# Autodesk Inventor assembly: Master
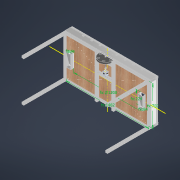
[picture p0: Inventor's stored thumbnail of the model, 180x180]
Saved by Autodesk Inventor 2021.4 (Build 254397000, 397)
## iProperties
Created: 2021-11-23
Part Number: Master
Document SubType Name: Assembly
Designer: jo_ki
Author: jo_ki
## Documents named in this file (35)
- D:\Repos\SmartSoccerTableCAD\Assemblies\Master.iam
- D:\Repos\SmartSoccerTableCAD\Parts\Beams\leg.ipt
- D:\Repos\SmartSoccerTableCAD\Parts\Beams\tallBeamLong.ipt
- D:\Repos\SmartSoccerTableCAD\Parts\Beams\tallBeamShort.ipt
- D:\Repos\SmartSoccerTableCAD\Parts\Beams\tallBeamLongInlet.ipt
- D:\Repos\SmartSoccerTableCAD\Parts\ballInlet\ballInletWheel.ipt
- D:\Repos\SmartSoccerTableCAD\Parts\Dimensions\Mastersketch.ipt
- D:\Repos\SmartSoccerTableCAD\Parts\Floors\GroundPlate.ipt
- D:\Repos\SmartSoccerTableCAD\Parts\Floors\glassPlate.ipt
- D:\Repos\SmartSoccerTableCAD\Parts\goalStructure\goalPanelFront.ipt
- D:\Repos\SmartSoccerTableCAD\Parts\goalStructure\goalPanelTop.ipt
- D:\Repos\SmartSoccerTableCAD\Parts\Beams\centerSupportBeam.ipt
- D:\Repos\SmartSoccerTableCAD\Import\stepper_am23hs0420-01\stepper_am23hs0420-01.iam
- D:\Repos\SmartSoccerTableCAD\Parts\Beams\centerAxleSupportBeam.ipt
- D:\Repos\SmartSoccerTableCAD\Parts\ballInlet\stepperMotorMount.ipt
- D:\Repos\SmartSoccerTableCAD\Parts\Beams\centerAxleSupportBeamHole.ipt
- D:\Repos\SmartSoccerTableCAD\Parts\ballInlet\axleMount\bearingShellInner.ipt
- D:\Repos\SmartSoccerTableCAD\Parts\ballInlet\axleMount\bearingShellOuter.ipt
- D:\Repos\SmartSoccerTableCAD\Parts\ballInlet\axleMount\centerAxleBearingSpacer.ipt
- C:\Users\jo_ki\OneDrive\Dokumente\Inventor\Content Center Files\R2021\en-US\DIN 625 SKF(4)\DIN 625 SKF - SKF 61800-2Z.ipt
- D:\Repos\SmartSoccerTableCAD\Parts\ballInlet\ballInletWheelAxle.ipt
- D:\Repos\SmartSoccerTableCAD\Parts\ballInlet\stepperToAxleConnector_1.ipt
- D:\Repos\SmartSoccerTableCAD\Parts\ballInlet\stepperToAxleConnector_2.ipt
- C:\Users\jo_ki\OneDrive\Dokumente\Inventor\Content Center Files\R2021\en-US\ISO 4762(2)\ISO 4762 - M3 x 6ISO.ipt
- C:\Users\jo_ki\OneDrive\Dokumente\Inventor\Content Center Files\R2021\en-US\ISO 4762(2)\ISO 4762 - M5 x 16ISO.ipt
- C:\Users\jo_ki\OneDrive\Dokumente\Inventor\Content Center Files\R2021\en-US\ISO 4035(2)\ISO 4035 - M10 - ISO.ipt
- C:\Users\jo_ki\OneDrive\Dokumente\Inventor\Content Center Files\R2021\en-US\ISO 7089\ISO 7089 - 10 - 140 HV(1).ipt
- D:\Repos\SmartSoccerTableCAD\Import\Nutenstein_8_St_M6\Nutenstein_8_St_M6.ipt
- C:\Users\jo_ki\OneDrive\Dokumente\Inventor\Content Center Files\R2021\en-US\ISO 4762(2)\ISO 4762 - M6 x 16ISO.ipt
- D:\Repos\SmartSoccerTableCAD\Parts\goalStructure\TorraumSeitenplatte.ipt
- D:\Repos\SmartSoccerTableCAD\Parts\goalStructure\TorraumSchrägeObenNEU.ipt
- D:\Repos\SmartSoccerTableCAD\Parts\goalStructure\TorraumHinten.ipt
- D:\Repos\SmartSoccerTableCAD\Parts\goalStructure\TorraumSchrägeUntenNEU.ipt
- D:\Repos\SmartSoccerTableCAD\Parts\goalStructure\TorraumSeiteBalleinwurf.ipt
- D:\Repos\SmartSoccerTableCAD\Parts\goalStructure\TorraumFrontKlein.ipt
## Components (53 placed, 33 different names)
1. glassPlate:1 — Mate:15, Mate:16, Flush:29, Mate:19, Mate:21
2. GroundPlate:1 — Mate:10, Mate:11, Mate:12, Mate:15, Flush:29, Mate:18, Mate:22, Mate:26, Mate:85
3. Nutenstein_8_St_M6:1 — Mate:80, Mate:81, Mate:82, Mate:83
4. ISO 4762 M6 x 16:1 — Mate:83, Mate:84
5. ISO 4762 M3 x 6:2 — Mate:62, Mate:63
6. ISO 4762 M3 x 6:3 — Mate:64, Mate:65
7. ISO 4762 M3 x 6:4 — Mate:66, Mate:67
8. ISO 4762 M5 x 16:1 — Mate:68, Mate:69
9. ISO 4762 M5 x 16:2 — Mate:70, Mate:71
10. ISO 4762 M5 x 16:3 — Mate:72, Mate:73
11. ISO 4762 M5 x 16:4 — Mate:74, Mate:75
12. ISO 7089 10:1 — Mate:76, Mate:77, Mate:79
13. ISO 4035 M10:1 — Mate:78, Mate:79, Angle:1
14. stepper_am23hs0420-01:1 [sub-assembly] — Flush:36, Flush:37, Mate:36, Mate:37, Mate:69, Mate:71, Mate:73, Mate:75
15. stepperMotorMount:1 — Mate:34, Mate:35, Flush:36, Flush:37, Mate:37, Mate:68, Mate:70, Mate:72, Mate:74, Mate:81, Mate:82, Mate:84
16. centerAxleSupportBeamHole:1 — Mate:38, Mate:39, Mate:40, Mate:41, Mate:50, Mate:51
17. bearingShellInner:1 — Mate:42, Mate:43, Mate:44, Mate:45, Mate:47
18. bearingShellOuter:1 — Mate:42, Mate:46, Mate:50, Mate:51
19. centerAxleBearingSpacer:1 — Mate:47, Mate:48, Mate:49
20. DIN 625 SKF- with two Z shields SKF 61800-2Z:1 — Mate:43, Mate:44, Mate:49
21. DIN 625 SKF- with two Z shields SKF 61800-2Z:2 — Mate:45, Mate:46, Mate:48
22. ballInletWheelAxle:1 — Mate:52, Mate:53, Mate:54, Mate:55, Mate:56, Mate:57, Mate:59, Mate:76, Mate:78, Angle:1
23. stepperToAxleConnector_1:1 — Flush:38, Mate:58, Mate:59, Mate:61, Mate:63, Mate:65, Mate:67
24. stepperToAxleConnector_2:1 — Mate:55, Mate:56, Mate:57, Flush:38, Mate:58, Mate:60, Mate:62, Mate:64, Mate:66
25. ISO 4762 M3 x 6:1 — Mate:60, Mate:61
26. centerSupportBeam:1 — Mate:29, Flush:32, Tangent:2, Mate:32, Flush:35, Mate:38
27. centerSupportBeam:2 — Mate:30, Flush:33, Tangent:1
28. centerAxleSupportBeam:1 — Mate:32, Flush:35, Mate:34, Mate:35, Mate:41, Mate:80
29. ballInletWheel:1 — Mate:9, Flush:17, Tangent:1, Tangent:2, Mate:36, Mate:39, Mate:40, Mate:52, Mate:53, Mate:54, Mate:77
30. leg:1 — Flush:1, Flush:23, Mate:14
31. leg:2 — Flush:14, Flush:15, Mate:8
32. leg:3 — Flush:3, Mate:13, Flush:21, Flush:22
33. leg:4 — Mate:6, Flush:12, Flush:13
34. tallBeamLong:1 — Flush:1, Flush:3, Mate:3, Mate:5, Mate:11, Flush:18, Flush:19, Flush:20, Mate:13, Flush:21, Mate:14, Mate:17, Mate:20, Mate:23, Mate:25
35. tallBeamShort:1 — Mate:5, Flush:15, Flush:16, Flush:20, Flush:22
36. tallBeamShort:2 — Mate:3, Flush:10, Mate:7, Flush:11, Flush:12, Mate:12, Flush:18, Flush:19, Flush:23
37. tallBeamLongInlet:1 — Mate:6, Flush:10, Mate:7, Flush:11, Flush:13, Flush:14, Flush:16, Mate:8, Mate:9, Flush:17, Mate:10, Mate:16, Mate:27, Mate:29, Flush:32, Mate:30, Flush:33
38. goalPanelFront:1 — Mate:17, Mate:18, Mate:19, Mate:26, Flush:31, Mate:28, Mate:86, Mate:88, Mate:90, Mate:99
39. TorraumSeitenplatte:1 — Mate:85, Mate:86, Mate:87, Mate:89, Flush:39, Flush:41
40. TorraumSchrägeObenNEU:1 — Mate:88, Mate:89, Mate:90, Mate:92
41. TorraumHinten:1 — Mate:91, Mate:92, Flush:39, Flush:40, Mate:93, Mate:94, Mate:95, Flush:42
42. TorraumSchrägeUntenNEU:1 — Flush:40, Mate:93, Mate:94, Mate:98
43. TorraumSeiteBalleinwurf:1 — Mate:95, Mate:97, Flush:42
44. TorraumFrontKlein:1 — Mate:98, Flush:41, Mate:99
45. goalPanelTop:1 — Mate:25, Mate:27, Flush:31, Mate:28, Mate:87, Mate:91, Mate:97
46. TorraumSeitenplatte:2 — Mate:110, Flush:45, Mate:111
47. TorraumFrontKlein:2 — Flush:43, Mate:106, Mate:107
48. TorraumHinten:2 — Mate:103, Mate:104, Mate:105, Mate:108, Flush:44, Mate:109, Mate:110, Flush:45, Mate:112
49. TorraumSchrägeObenNEU:2 — Mate:112, Mate:113, Mate:114
50. TorraumSchrägeUntenNEU:2 — Mate:108, Flush:44, Mate:109
51. TorraumSeiteBalleinwurf:2 — Mate:100, Mate:101, Mate:102, Mate:103, Mate:104, Mate:107, Mate:114
52. goalPanelTop:2 — Mate:23, Mate:24, Flush:30, Mate:101, Mate:105, Mate:111
53. goalPanelFront:2 — Mate:20, Mate:21, Mate:22, Mate:24, Flush:30, Mate:100, Mate:102, Flush:43, Mate:106, Mate:113
## Relationships (143: Mate 108, Flush 32, Tangent 2, Angle 1)
- Flush:1: leg:1 ↔ tallBeamLong:1
- Flush:3: leg:3 ↔ tallBeamLong:1
- Mate:3: tallBeamLong:1 ↔ tallBeamShort:2
- Mate:5: tallBeamLong:1 ↔ tallBeamShort:1
- Mate:6: leg:4 ↔ tallBeamLongInlet:1
- Flush:10: tallBeamShort:2 ↔ tallBeamLongInlet:1
- Mate:7: tallBeamShort:2 ↔ tallBeamLongInlet:1
- Flush:11: tallBeamShort:2 ↔ tallBeamLongInlet:1
- Flush:12: leg:4 ↔ tallBeamShort:2
- Flush:13: leg:4 ↔ tallBeamLongInlet:1
- Flush:14: leg:2 ↔ tallBeamLongInlet:1
- Flush:15: leg:2 ↔ tallBeamShort:1
- Flush:16: tallBeamShort:1 ↔ tallBeamLongInlet:1
- Mate:8: leg:2 ↔ tallBeamLongInlet:1
- Mate:9: ballInletWheel:1 ↔ tallBeamLongInlet:1
- Flush:17 (4.5 mm): ballInletWheel:1 ↔ tallBeamLongInlet:1
- Mate:10: GroundPlate:1 ↔ tallBeamLongInlet:1
- Mate:11 (-11 mm): GroundPlate:1 ↔ tallBeamLong:1
- Mate:12 (-11 mm): GroundPlate:1 ↔ tallBeamShort:2
- Flush:18: tallBeamLong:1 ↔ tallBeamShort:2
- Flush:19: tallBeamLong:1 ↔ tallBeamShort:2
- Flush:20: tallBeamLong:1 ↔ tallBeamShort:1
- Mate:13: leg:3 ↔ tallBeamLong:1
- Flush:21: leg:3 ↔ tallBeamLong:1
- Flush:22: leg:3 ↔ tallBeamShort:1
- Flush:23: leg:1 ↔ tallBeamShort:2
- Mate:14: leg:1 ↔ tallBeamLong:1
- Mate:15: glassPlate:1 ↔ GroundPlate:1
- Mate:16: glassPlate:1 ↔ tallBeamLongInlet:1
- Flush:29: glassPlate:1 ↔ GroundPlate:1
- Mate:17: tallBeamLong:1 ↔ goalPanelFront:1
- Mate:18: GroundPlate:1 ↔ goalPanelFront:1
- Mate:19: glassPlate:1 ↔ goalPanelFront:1
- Mate:20: tallBeamLong:1 ↔ goalPanelFront:2
- Mate:21: glassPlate:1 ↔ goalPanelFront:2
- Mate:22: GroundPlate:1 ↔ goalPanelFront:2
- Mate:23: tallBeamLong:1 ↔ goalPanelTop:2
- Mate:24: goalPanelTop:2 ↔ goalPanelFront:2
- Flush:30: goalPanelTop:2 ↔ goalPanelFront:2
- Mate:25: tallBeamLong:1 ↔ goalPanelTop:1
- Mate:26: GroundPlate:1 ↔ goalPanelFront:1
- Mate:27: tallBeamLongInlet:1 ↔ goalPanelTop:1
- Flush:31: goalPanelFront:1 ↔ goalPanelTop:1
- Mate:28: goalPanelFront:1 ↔ goalPanelTop:1
- Mate:29: centerSupportBeam:1 ↔ tallBeamLongInlet:1
- Flush:32: centerSupportBeam:1 ↔ tallBeamLongInlet:1
- Mate:30: centerSupportBeam:2 ↔ tallBeamLongInlet:1
- Flush:33: centerSupportBeam:2 ↔ tallBeamLongInlet:1
- Tangent:1 (10 mm): centerSupportBeam:2 ↔ ballInletWheel:1
- Tangent:2 (10 mm): centerSupportBeam:1 ↔ ballInletWheel:1
- Mate:32: centerSupportBeam:1 ↔ centerAxleSupportBeam:1
- Flush:35: centerSupportBeam:1 ↔ centerAxleSupportBeam:1
- Mate:34: stepperMotorMount:1 ↔ centerAxleSupportBeam:1
- Mate:35: stepperMotorMount:1 ↔ centerAxleSupportBeam:1
- Flush:36: stepper_am23hs0420-01:1 ↔ stepperMotorMount:1
- Flush:37: stepper_am23hs0420-01:1 ↔ stepperMotorMount:1
- Mate:36: stepper_am23hs0420-01:1 ↔ ballInletWheel:1
- Mate:37: stepper_am23hs0420-01:1 ↔ stepperMotorMount:1
- Mate:38: centerAxleSupportBeamHole:1 ↔ centerSupportBeam:1
- Mate:39: centerAxleSupportBeamHole:1 ↔ ballInletWheel:1
- Mate:40 (10 mm): centerAxleSupportBeamHole:1 ↔ ballInletWheel:1
- Mate:41 (200 mm): centerAxleSupportBeamHole:1 ↔ centerAxleSupportBeam:1
- Mate:42: bearingShellInner:1 ↔ bearingShellOuter:1
- Mate:43: bearingShellInner:1 ↔ DIN 625 SKF- with two Z shields SKF 61800-2Z:1
- Mate:44: bearingShellInner:1 ↔ DIN 625 SKF- with two Z shields SKF 61800-2Z:1
- Mate:45: bearingShellInner:1 ↔ DIN 625 SKF- with two Z shields SKF 61800-2Z:2
- Mate:46: bearingShellOuter:1 ↔ DIN 625 SKF- with two Z shields SKF 61800-2Z:2
- Mate:47: bearingShellInner:1 ↔ centerAxleBearingSpacer:1
- Mate:48: centerAxleBearingSpacer:1 ↔ DIN 625 SKF- with two Z shields SKF 61800-2Z:2
- Mate:49: centerAxleBearingSpacer:1 ↔ DIN 625 SKF- with two Z shields SKF 61800-2Z:1
- Mate:50: centerAxleSupportBeamHole:1 ↔ bearingShellOuter:1
- Mate:51: centerAxleSupportBeamHole:1 ↔ bearingShellOuter:1
- Mate:52: ballInletWheelAxle:1 ↔ ballInletWheel:1
- Mate:53: ballInletWheelAxle:1 ↔ ballInletWheel:1
- Mate:54: ballInletWheelAxle:1 ↔ ballInletWheel:1
- Mate:55: ballInletWheelAxle:1 ↔ stepperToAxleConnector_2:1
- Mate:56: ballInletWheelAxle:1 ↔ stepperToAxleConnector_2:1
- Mate:57 (2.5 mm): ballInletWheelAxle:1 ↔ stepperToAxleConnector_2:1
- Flush:38: stepperToAxleConnector_1:1 ↔ stepperToAxleConnector_2:1
- Mate:58: stepperToAxleConnector_1:1 ↔ stepperToAxleConnector_2:1
- Mate:59: ballInletWheelAxle:1 ↔ stepperToAxleConnector_1:1
- Mate:60: stepperToAxleConnector_2:1 ↔ ISO 4762 M3 x 6:1
- Mate:61: stepperToAxleConnector_1:1 ↔ ISO 4762 M3 x 6:1
- Mate:62: ISO 4762 M3 x 6:2 ↔ stepperToAxleConnector_2:1
- Mate:63: ISO 4762 M3 x 6:2 ↔ stepperToAxleConnector_1:1
- Mate:64: ISO 4762 M3 x 6:3 ↔ stepperToAxleConnector_2:1
- Mate:65: ISO 4762 M3 x 6:3 ↔ stepperToAxleConnector_1:1
- Mate:66: ISO 4762 M3 x 6:4 ↔ stepperToAxleConnector_2:1
- Mate:67: ISO 4762 M3 x 6:4 ↔ stepperToAxleConnector_1:1
- Mate:68: ISO 4762 M5 x 16:1 ↔ stepperMotorMount:1
- Mate:69: ISO 4762 M5 x 16:1 ↔ stepper_am23hs0420-01:1
- Mate:70: ISO 4762 M5 x 16:2 ↔ stepperMotorMount:1
- Mate:71: ISO 4762 M5 x 16:2 ↔ stepper_am23hs0420-01:1
- Mate:72: ISO 4762 M5 x 16:3 ↔ stepperMotorMount:1
- Mate:73: ISO 4762 M5 x 16:3 ↔ stepper_am23hs0420-01:1
- Mate:74: ISO 4762 M5 x 16:4 ↔ stepperMotorMount:1
- Mate:75: ISO 4762 M5 x 16:4 ↔ stepper_am23hs0420-01:1
- Mate:76: ISO 7089 10:1 ↔ ballInletWheelAxle:1
- Mate:77: ISO 7089 10:1 ↔ ballInletWheel:1
- Mate:78: ISO 4035 M10:1 ↔ ballInletWheelAxle:1
- Mate:79: ISO 7089 10:1 ↔ ISO 4035 M10:1
- Angle:1 (0 deg): ISO 4035 M10:1 ↔ ballInletWheelAxle:1
- Mate:80: Nutenstein_8_St_M6:1 ↔ centerAxleSupportBeam:1
- Mate:81: Nutenstein_8_St_M6:1 ↔ stepperMotorMount:1
- Mate:82 (1 mm): Nutenstein_8_St_M6:1 ↔ stepperMotorMount:1
- Mate:83: Nutenstein_8_St_M6:1 ↔ ISO 4762 M6 x 16:1
- Mate:84: ISO 4762 M6 x 16:1 ↔ stepperMotorMount:1
- Mate:85: GroundPlate:1 ↔ TorraumSeitenplatte:1
- Mate:86: goalPanelFront:1 ↔ TorraumSeitenplatte:1
- Mate:87: TorraumSeitenplatte:1 ↔ goalPanelTop:1
- Mate:88: goalPanelFront:1 ↔ TorraumSchrägeObenNEU:1
- Mate:89: TorraumSeitenplatte:1 ↔ TorraumSchrägeObenNEU:1
- Mate:90: goalPanelFront:1 ↔ TorraumSchrägeObenNEU:1
- Mate:91: TorraumHinten:1 ↔ goalPanelTop:1
- Mate:92: TorraumSchrägeObenNEU:1 ↔ TorraumHinten:1
- Flush:39: TorraumSeitenplatte:1 ↔ TorraumHinten:1
- Flush:40: TorraumHinten:1 ↔ TorraumSchrägeUntenNEU:1
- Mate:93: TorraumHinten:1 ↔ TorraumSchrägeUntenNEU:1
- Mate:94: TorraumHinten:1 ↔ TorraumSchrägeUntenNEU:1
- Mate:95: TorraumHinten:1 ↔ TorraumSeiteBalleinwurf:1
- Mate:97: TorraumSeiteBalleinwurf:1 ↔ goalPanelTop:1
- Mate:98: TorraumSchrägeUntenNEU:1 ↔ TorraumFrontKlein:1
- Flush:41: TorraumSeitenplatte:1 ↔ TorraumFrontKlein:1
- Mate:99: goalPanelFront:1 ↔ TorraumFrontKlein:1
- Flush:42: TorraumHinten:1 ↔ TorraumSeiteBalleinwurf:1
- Mate:100: TorraumSeiteBalleinwurf:2 ↔ goalPanelFront:2
- Mate:101: TorraumSeiteBalleinwurf:2 ↔ goalPanelTop:2
- Mate:102: TorraumSeiteBalleinwurf:2 ↔ goalPanelFront:2
- Mate:103: TorraumHinten:2 ↔ TorraumSeiteBalleinwurf:2
- Mate:104: TorraumHinten:2 ↔ TorraumSeiteBalleinwurf:2
- Mate:105: TorraumHinten:2 ↔ goalPanelTop:2
- Flush:43: TorraumFrontKlein:2 ↔ goalPanelFront:2
- Mate:106: TorraumFrontKlein:2 ↔ goalPanelFront:2
- Mate:107: TorraumFrontKlein:2 ↔ TorraumSeiteBalleinwurf:2
- Mate:108: TorraumHinten:2 ↔ TorraumSchrägeUntenNEU:2
- Flush:44: TorraumHinten:2 ↔ TorraumSchrägeUntenNEU:2
- Mate:109: TorraumHinten:2 ↔ TorraumSchrägeUntenNEU:2
- Mate:110: TorraumSeitenplatte:2 ↔ TorraumHinten:2
- Flush:45: TorraumSeitenplatte:2 ↔ TorraumHinten:2
- Mate:111: TorraumSeitenplatte:2 ↔ goalPanelTop:2
- Mate:112: TorraumHinten:2 ↔ TorraumSchrägeObenNEU:2
- Mate:113: TorraumSchrägeObenNEU:2 ↔ goalPanelFront:2
- Mate:114: TorraumSchrägeObenNEU:2 ↔ TorraumSeiteBalleinwurf:2
## Named parameters: profile_width = 40 mm, feet_widthCenter = 720 mm, feet_lengthCenter = 1500 mm, feet_length = 746 mm, profile_height = 160 mm, groundPlate_width = 702 mm, groundPlate_length = 1482 mm, handle_distance = 150 mm, handle_amount = 8, handle_offsetTop = 45 mm, handleAxle_diameter = 16 mm, handleHole_diameter = 36 mm, profileTall_innerHeightOffset = 33 mm, profileTallWall_thickness = 3 mm, groundPlate_thickness = 8 mm, ball_size = 33 mm, ball_rollTolerance = 1 mm, glass_thickness = 6 mm, glass_length = 1200 mm, ballInletHole_groundPlateOffsetBottom = 24 mm, ballInletWheel_margin = 10 mm, ballInletWheel_thickness = 31 mm, ballInletWheelBucket_amount = 6, ballInletWheelSlope_angle = 10 deg, goal_width = 224 mm, goal_height = 96 mm, goal_depth = 84 mm, goalCollector_depth = 68 mm, ballRollbackRail_angle = 5 deg, handleAxle_length = 1100 mm, ballInletWheelDriveShaftAxle_diameter = 10 mm, ballInletWheel_diameter = 238.29764 mm, ballInletWheel_offsetTop = 174.68268 mm, ballInletWheel_tolerance = 1 mm, ballInletHole_bottomOffset = 71.5 mm, playAreaWall_height = 130 mm, goalPanel_thickness = 4 mm, goalArea_width = 130 mm, goalCollector_angle = 45 deg, goalCollectorRollback_angle = 45 deg, goalPlayArea_distance = 228 mm, goalPanelFrontInner_innerWidth = 220 mm, goalPanelBackInner_innerWidth = 672 mm, goalPanelSideOuter_width = 141 mm, goalCollectorPanelSide_angel = 45 deg, goalCollectorRollbackPipe_diameter = 35 mm, pipeConnector_wallThickness = 3 mm, pipe_wallThickness = 2 mm, axleSupport_offset = 14.68268 mm, axleSupport_distance = 200 mm
